# Autodesk Inventor assembly: Butterfly Drive Module
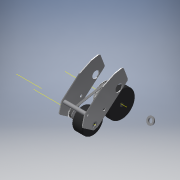
[picture p0: Inventor's stored thumbnail of the model, 180x180]
Saved by Autodesk Inventor 2019 (Build 230136000, 136)
## iProperties
Created: 2019-10-18
Part Number: Butterfly Drive Module
Document SubType Name: Assembly
Designer: admin
Author: admin
## Documents named in this file (8)
- C:\Users\Mark\Desktop\7738 Helion Engineering\7738-CAD-prep\Butterfly drive\Butterfly Drive Module.iam
- C:\Users\Mark\Desktop\7738 Helion Engineering\7738-CAD-prep\Butterfly drive\100mm Mecanum StandIn.ipt
- C:\Users\Mark\Desktop\7738 Helion Engineering\7738-CAD-prep\Butterfly drive\100mm Traction Wheel StandIn.ipt
- C:\Users\Mark\Desktop\7738 Helion Engineering\7738-CAD-prep\Butterfly drive\Butterfly Drive Module\Design Accelerator\Synchronous Belts Transmission3.iam
- C:\Users\Mark\Desktop\7738 Helion Engineering\7738-CAD-prep\Butterfly drive\Module Plate 1.ipt
- C:\Users\Mark\Desktop\7738 Helion Engineering\7738-CAD-prep\Butterfly drive\Connector.ipt
- C:\Users\Mark\Desktop\7738 Helion Engineering\7738-CAD-prep\Butterfly drive\F6004.ipt
- C:\Users\Mark\Desktop\7738 Helion Engineering\7738-CAD-prep\Butterfly drive\F6802.ipt
## Components (11 placed, 7 different names)
1. Connector:1 — Mate:34, Insert:5
2. 100mm Mecanum StandIn:1 — Flush:1, Mate:5, Angle:1, Mate:37, Mate:42
3. 100mm Traction Wheel StandIn:1 — Mate:4, Flush:1, Mate:6
4. Synchronous Belts Transmission:1 [sub-assembly] — Mate:5, Mate:6, Mate:37, Mate:40, Mate:41, Mate:45
5. Module Plate 1:1 — Mate:33, Flush:2, Flush:3, Insert:3, Insert:5, Mate:39, Mate:41, Mate:42, Rotational:2, Mate:43, Mate:44
6. Module Plate 1:2 — Mate:33, Flush:2, Flush:3, Insert:4, Rotational:1
7. F6804:1 — Rotational:1
8. F6804:2 — Rotational:2
9. F6802:1 — Insert:4
10. F6802:2 — Insert:3, Mate:45
11. Connector:2 — Mate:43, Mate:44
## Relationships (22: Mate 13, Flush 3, Insert 3, RevoluteJoint 2, Angle 1)
- Mate:4: 100mm Traction Wheel StandIn:1
- Flush:1 (10 mm): 100mm Mecanum StandIn:1 ↔ 100mm Traction Wheel StandIn:1
- Mate:5: 100mm Mecanum StandIn:1 ↔ Synchronous Belts Transmission:1
- Mate:6: 100mm Traction Wheel StandIn:1 ↔ Synchronous Belts Transmission:1
- Angle:1 (90 deg): 100mm Mecanum StandIn:1
- Mate:33 (105 mm): Module Plate 1:1 ↔ Module Plate 1:2
- Mate:34: Connector:1
- Flush:2: Module Plate 1:1 ↔ Module Plate 1:2
- Flush:3: Module Plate 1:1 ↔ Module Plate 1:2
- Mate:37 (2 mm): 100mm Mecanum StandIn:1 ↔ Synchronous Belts Transmission:1
- Insert:3: Module Plate 1:1 ↔ F6802:2
- Insert:4: Module Plate 1:2 ↔ F6802:1
- Insert:5: Connector:1 ↔ Module Plate 1:1
- Mate:39: Module Plate 1:1
- Mate:40: Synchronous Belts Transmission:1
- Mate:41: Synchronous Belts Transmission:1 ↔ Module Plate 1:1
- Mate:42 (3.5 mm): 100mm Mecanum StandIn:1 ↔ Module Plate 1:1
- Rotational:1 [RevoluteJoint]: Module Plate 1:2 ↔ F6804:1
- Rotational:2 [RevoluteJoint]: Module Plate 1:1 ↔ F6804:2
- Mate:43: Module Plate 1:1 ↔ Connector:2
- Mate:44: Module Plate 1:1 ↔ Connector:2
- Mate:45: Synchronous Belts Transmission:1 ↔ F6802:2
